# Autodesk Inventor assembly: Carriage_Assembly
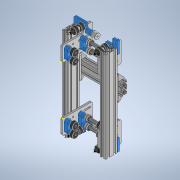
[picture p0: Inventor's stored thumbnail of the model, 180x180]
Saved by Autodesk Inventor 2021 (Build 250183000, 183)
## iProperties
Created: 2021-09-08
Part Number: Carriage_Assembly
Document SubType Name: Assembly
Designer: Jorian Brusind
Author: Jorian Brusind
## Documents named in this file (11)
- C:\Users\Jorian Brusind\Documents\GitHub\PersonalProjects\HyperRail\Inventor Files\Carriage_Assembly.iam
- C:\Users\Jorian Brusind\Documents\GitHub\PersonalProjects\Inventor Projects\Useful models\8020_Sets\IPT_20_Series\IPT_20_Series\20-2040_150mm.ipt
- C:\Users\Jorian Brusind\Documents\GitHub\PersonalProjects\HyperRail\Inventor Files\X_CarriageL_V2_0_Short.iam
- C:\Users\Jorian Brusind\Documents\GitHub\PersonalProjects\HyperRail\Inventor Files\X_CarriageR_V2_0_Short.iam
- C:\Users\Jorian Brusind\Documents\GitHub\PersonalProjects\HyperRail\Inventor Files\X_CarriageR_V2_0.iam
- C:\Users\Jorian Brusind\Documents\GitHub\PersonalProjects\HyperRail\Inventor Files\X_Carriage_V2_0.iam
- C:\Users\Jorian Brusind\Documents\GitHub\PersonalProjects\Inventor Projects\Useful models\8020_Sets\IPT_20_Series\Extra_20_Series\8020_14056m\14056_m.ipt
- C:\Users\Jorian Brusind\Documents\GitHub\PersonalProjects\HyperRail\Inventor Files\Buffer.iam
- C:\Users\Jorian Brusind\Documents\GitHub\PersonalProjects\Inventor Projects\Useful models\Metric Spacer_Standoffs\hex spacer standoff nut M5 L30.ipt
- C:\Users\Jorian Brusind\Documents\GitHub\PersonalProjects\HyperRail\Inventor Files\Carriage_Horizontal_Spacer.ipt
- C:\Users\Jorian Brusind\Documents\GitHub\PersonalProjects\Inventor Projects\Useful models\8020_Sets\IPT_20_Series\IPT_20_Series\20-2040_400mm.ipt
## Components (21 placed, 10 different names)
1. 20-2040_150mm:1 — Mate:8, Mate:20, Mate:21, Mate:22, Mate:23, Mate:80, Flush:33
2. X_CarriageL_V2_0_Short:1 [sub-assembly] — Mate:57, Mate:65, Mate:68, Mate:81, Mate:83
3. X_CarriageR_V2_0_Short:1 [sub-assembly] — Mate:59, Mate:60, Mate:63, Mate:85, Flush:40
4. X_CarriageR_V2_0:1 [sub-assembly] — Mate:8, Mate:54, Mate:64, Mate:66, Mate:67, Flush:31, Mate:78, Flush:32, Flush:34
5. X_Carriage_V2_0:1 [sub-assembly] — Mate:55, Mate:58, Mate:61, Mate:62, Mate:77, Flush:31, Flush:32, Flush:35, Flush:40
6. 14056_m:1 — Mate:21, Flush:26, Flush:38
7. 14056_m:2 — Mate:20, Flush:25, Flush:26, Mate:70, Flush:37, Flush:39
8. 14056_m:3 — Mate:22, Flush:13
9. 14056_m:4 — Mate:23, Flush:13, Flush:28, Mate:72
10. Buffer:1 [sub-assembly] — Mate:57, Mate:82, Flush:41
11. Buffer:2 [sub-assembly] — Mate:54, Mate:86
12. Buffer:3 [sub-assembly] — Flush:42, Mate:87, Flush:43
13. Buffer:4 [sub-assembly] — Mate:55, Mate:88
14. hex spacer standoff nut M5 L30:2 — Mate:64, Mate:65, Mate:66
15. hex spacer standoff nut M5 L30:3 — Mate:67, Mate:68
16. hex spacer standoff nut M5 L30:4 — Mate:62, Mate:63
17. hex spacer standoff nut M5 L30:6 — Mate:58, Mate:59, Mate:60, Mate:61
18. Carriage_Horizontal_Spacer:1 — Flush:28, Mate:72, Mate:79, Mate:80
19. Carriage_Horizontal_Spacer:2 — Flush:25, Mate:70, Mate:84, Flush:37, Flush:38
20. 20-2040_400mm:1 — Flush:30, Mate:75, Mate:76, Mate:77, Mate:78, Mate:79, Flush:33, Flush:34, Flush:35, Flush:36, Mate:86, Mate:88
21. 20-2040_400mm:2 — Flush:30, Mate:81, Flush:36, Mate:82, Mate:83, Mate:84, Mate:85, Flush:39, Flush:41, Flush:42, Mate:87, Flush:43
## Relationships (53: Mate 35, Flush 18)
- Mate:8 (30 mm): 20-2040_150mm:1 ↔ X_CarriageR_V2_0:1
- Mate:20: 20-2040_150mm:1 ↔ 14056_m:2
- Mate:21: 20-2040_150mm:1 ↔ 14056_m:1
- Mate:22: 20-2040_150mm:1 ↔ 14056_m:3
- Mate:23: 20-2040_150mm:1 ↔ 14056_m:4
- Flush:13: 14056_m:3 ↔ 14056_m:4
- Mate:54: X_CarriageR_V2_0:1 ↔ Buffer:2
- Mate:55: X_Carriage_V2_0:1 ↔ Buffer:4
- Mate:57: X_CarriageL_V2_0_Short:1 ↔ Buffer:1
- Mate:58: X_Carriage_V2_0:1 ↔ hex spacer standoff nut M5 L30:6
- Mate:59: X_CarriageR_V2_0_Short:1 ↔ hex spacer standoff nut M5 L30:6
- Mate:60: X_CarriageR_V2_0_Short:1 ↔ hex spacer standoff nut M5 L30:6
- Mate:61: X_Carriage_V2_0:1 ↔ hex spacer standoff nut M5 L30:6
- Mate:62: X_Carriage_V2_0:1 ↔ hex spacer standoff nut M5 L30:4
- Mate:63: X_CarriageR_V2_0_Short:1 ↔ hex spacer standoff nut M5 L30:4
- Mate:64: X_CarriageR_V2_0:1 ↔ hex spacer standoff nut M5 L30:2
- Mate:65: X_CarriageL_V2_0_Short:1 ↔ hex spacer standoff nut M5 L30:2
- Mate:66: X_CarriageR_V2_0:1 ↔ hex spacer standoff nut M5 L30:2
- Mate:67: X_CarriageR_V2_0:1 ↔ hex spacer standoff nut M5 L30:3
- Mate:68: X_CarriageL_V2_0_Short:1 ↔ hex spacer standoff nut M5 L30:3
- Flush:25: 14056_m:2 ↔ Carriage_Horizontal_Spacer:2
- Flush:26: 14056_m:1 ↔ 14056_m:2
- Mate:70: 14056_m:2 ↔ Carriage_Horizontal_Spacer:2
- Flush:28: 14056_m:4 ↔ Carriage_Horizontal_Spacer:1
- Mate:72: 14056_m:4 ↔ Carriage_Horizontal_Spacer:1
- Flush:30: 20-2040_400mm:1 ↔ 20-2040_400mm:2
- Mate:75: 20-2040_400mm:1
- Mate:76: 20-2040_400mm:1
- Mate:77: X_Carriage_V2_0:1 ↔ 20-2040_400mm:1
- Flush:31: X_CarriageR_V2_0:1 ↔ X_Carriage_V2_0:1
- Mate:78 (6 mm): X_CarriageR_V2_0:1 ↔ 20-2040_400mm:1
- Flush:32: X_CarriageR_V2_0:1 ↔ X_Carriage_V2_0:1
- Mate:79: Carriage_Horizontal_Spacer:1 ↔ 20-2040_400mm:1
- Mate:80: 20-2040_150mm:1 ↔ Carriage_Horizontal_Spacer:1
- Flush:33: 20-2040_150mm:1 ↔ 20-2040_400mm:1
- Flush:34: X_CarriageR_V2_0:1 ↔ 20-2040_400mm:1
- Flush:35: X_Carriage_V2_0:1 ↔ 20-2040_400mm:1
- Mate:81: X_CarriageL_V2_0_Short:1 ↔ 20-2040_400mm:2
- Flush:36: 20-2040_400mm:1 ↔ 20-2040_400mm:2
- Mate:82: Buffer:1 ↔ 20-2040_400mm:2
- Mate:83 (6 mm): X_CarriageL_V2_0_Short:1 ↔ 20-2040_400mm:2
- Mate:84: Carriage_Horizontal_Spacer:2 ↔ 20-2040_400mm:2
- Flush:37: 14056_m:2 ↔ Carriage_Horizontal_Spacer:2
- Flush:38: 14056_m:1 ↔ Carriage_Horizontal_Spacer:2
- Mate:85: X_CarriageR_V2_0_Short:1 ↔ 20-2040_400mm:2
- Flush:39: 14056_m:2 ↔ 20-2040_400mm:2
- Flush:40: X_CarriageR_V2_0_Short:1 ↔ X_Carriage_V2_0:1
- Mate:86: Buffer:2 ↔ 20-2040_400mm:1
- Flush:41: Buffer:1 ↔ 20-2040_400mm:2
- Flush:42: Buffer:3 ↔ 20-2040_400mm:2
- Mate:87: Buffer:3 ↔ 20-2040_400mm:2
- Flush:43: Buffer:3 ↔ 20-2040_400mm:2
- Mate:88: Buffer:4 ↔ 20-2040_400mm:1
